# Autodesk Inventor assembly: Assembly1
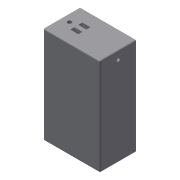
[picture p0: Inventor's stored thumbnail of the model, 180x180]
Saved by Autodesk Inventor 2016 SP2 (Build 200236200, 236)
## iProperties
Created: 2017-04-16
Part Number: Assembly1
Document SubType Name: Assembly
Designer: Karl
Author: Karl
## Documents named in this file (3)
- C:\Users\Karl\Desktop\LED Badge\CAD\Power Supply Case\Assembly1.iam
- C:\Users\Karl\Desktop\LED Badge\CAD\Power Supply Case\Case.ipt
- C:\Users\Karl\Desktop\LED Badge\CAD\Power Supply Case\Lid.ipt
## Components (2 placed, 2 different names)
1. Case:1 — Mate:1, Mate:2, Mate:3
2. Lid:1 — Mate:1, Mate:2, Mate:3
## Relationships (3: Mate 3)
- Mate:1: Case:1 ↔ Lid:1
- Mate:2: Case:1 ↔ Lid:1
- Mate:3: Case:1 ↔ Lid:1
